# Autodesk Inventor assembly: Behavioural Device assembly
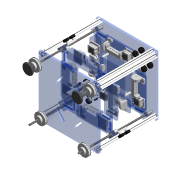
[picture p0: Inventor's stored thumbnail of the model, 180x180]
Saved by Autodesk Inventor 2020 (Build 240168000, 168)
## iProperties
Created: 2020-08-17
Part Number: Behavioural Device assembly
Document SubType Name: Assembly
Designer: ferrerx
Author: ferrerx
## Documents named in this file (22)
- C:\Users\ferrerx\Desktop\Prieto-Godino Lab\Drosophila Larvae Behavioural Device\Device design V3\Inventor Assembly\Behavioural Device assembly.iam
- C:\Users\ferrerx\Desktop\Inverted pendulum\aluminum profile.ipt
- C:\Users\ferrerx\Desktop\Prieto-Godino Lab\Drosophila Larvae Behavioural Device\Device design V3\Inventor Assembly\Z stage Base.ipt
- C:\Users\ferrerx\Desktop\Prieto-Godino Lab\Drosophila Larvae Behavioural Device\Device design V3\Inventor Assembly\Cart.ipt
- C:\Users\ferrerx\Desktop\Prieto-Godino Lab\Drosophila Larvae Behavioural Device\Device design V3\Inventor Assembly\Big pulley.ipt
- C:\Users\ferrerx\Desktop\Prieto-Godino Lab\Drosophila Larvae Behavioural Device\Device design V3\Inventor Assembly\guide wheel.ipt
- C:\Users\ferrerx\Desktop\Prieto-Godino Lab\Drosophila Larvae Behavioural Device\Device design V3\Inventor Assembly\Shaft connector.ipt
- C:\Users\ferrerx\Desktop\Prieto-Godino Lab\Drosophila Larvae Behavioural Device\Device design V3\Inventor Assembly\cart_spacer.ipt
- C:\Users\ferrerx\Desktop\Prieto-Godino Lab\Drosophila Larvae Behavioural Device\Device design V3\Inventor Assembly\Lead screw.ipt
- C:\Users\ferrerx\Desktop\Prieto-Godino Lab\Drosophila Larvae Behavioural Device\Device design V3\Inventor Assembly\lead screw nut.ipt
- C:\Users\ferrerx\Desktop\Prieto-Godino Lab\Drosophila Larvae Behavioural Device\Device design V3\Inventor Assembly\Light sources platform.ipt
- C:\Users\ferrerx\Desktop\Prieto-Godino Lab\Drosophila Larvae Behavioural Device\Device design V3\Inventor Assembly\Lead screw manual adjuster.ipt
- C:\Users\ferrerx\Desktop\Prieto-Godino Lab\Drosophila Larvae Behavioural Device\Device design V3\Inventor Assembly\Z stage Roof 2.ipt
- C:\Users\ferrerx\Desktop\Prieto-Godino Lab\Drosophila Larvae Behavioural Device\Device design V3\Inventor Assembly\Arena.ipt
- C:\Users\ferrerx\Desktop\Prieto-Godino Lab\Drosophila Larvae Behavioural Device\Device design V3\Inventor Assembly\Arena spacer.ipt
- C:\Users\ferrerx\Desktop\Prieto-Godino Lab\Drosophila Larvae Behavioural Device\Device design V3\Inventor Assembly\IR linear array assembly.iam
- C:\Users\ferrerx\Desktop\Prieto-Godino Lab\Drosophila Larvae Behavioural Device\Device design V3\Inventor Assembly\RGB matrices assembly.iam
- C:\Users\ferrerx\Desktop\Prieto-Godino Lab\Drosophila Larvae Behavioural Device\Device design V3\Inventor Assembly\Linear actuator assem 1.iam
- C:\Users\ferrerx\Desktop\Prieto-Godino Lab\Drosophila Larvae Behavioural Device\Device design V3\Inventor Assembly\pi_camera.ipt
- C:\Users\ferrerx\Desktop\Prieto-Godino Lab\Drosophila Larvae Behavioural Device\Device design V3\Inventor Assembly\Belt.ipt
- C:\Users\ferrerx\Desktop\Prieto-Godino Lab\Drosophila Larvae Behavioural Device\Device design V3\Inventor Assembly\LED Matrix Dotstar.ipt
- C:\Users\ferrerx\Desktop\Prieto-Godino Lab\Drosophila Larvae Behavioural Device\Device design V3\Inventor Assembly\LED Matrix 8X8.ipt
## Components (89 placed, 21 different names)
1. aluminum profile:1 — Mate:7, Mate:8, Mate:9, Mate:102, Mate:103, Mate:104, Angle:2, Angle:3
2. aluminum profile:2 — Mate:1, Mate:2, Mate:3, Angle:5
3. Z stage Base:2 — Mate:1, Mate:2, Mate:3, Mate:4, Mate:5, Mate:6, Mate:7, Mate:8, Mate:9, Mate:10, Mate:11, Mate:12, Mate:75, Mate:76, Mate:77, Mate:78, Mate:145, Mate:146, Mate:147, Mate:148, Mate:172, Mate:173, Mate:174, Mate:175, Mate:243, Mate:244
4. aluminum profile:3 — Mate:10, Mate:11, Mate:12, Angle:4
5. aluminum profile:4 — Mate:4, Mate:5, Mate:6, Angle:1, Angle:6
6. Cart:1 — Mate:45, Mate:46, Mate:47, Mate:48, Mate:49, Mate:50, Mate:52, Mate:53, Mate:69, Mate:70, Mate:87, Angle:4, Mate:196
7. Cart:2 — Mate:56, Mate:57, Mate:58, Mate:59, Mate:61, Mate:62, Mate:63, Mate:64, Mate:71, Mate:72, Mate:89, Mate:195, Angle:5
8. Big pulley:1 — Mate:95, Mate:106
9. Big pulley:2 — Mate:94, Mate:105, Mate:251, Mate:252
10. guide wheel:1 — Mate:29, Mate:55
11. guide wheel:2 — Mate:37, Mate:38
12. guide wheel:3 — Mate:44, Mate:60
13. guide wheel:4 — Mate:31, Mate:80
14. guide wheel:5 — Mate:32, Mate:51
15. guide wheel:6 — Mate:40, Mate:42
16. guide wheel:7 — Mate:30, Mate:54
17. guide wheel:8 — Mate:41, Mate:43
18. Shaft connector:1 — Mate:75, Mate:76, Mate:79, Mate:81
19. Shaft connector:2 — Mate:77, Mate:78, Mate:82, Mate:83
20. cart_spacer:1 — Mate:41, Mate:43, Mate:57, Mate:61
21. cart_spacer:2 — Mate:40, Mate:42, Mate:56, Mate:62
22. cart_spacer:3 — Mate:37, Mate:38, Mate:58, Mate:63
23. cart_spacer:4 — Mate:44, Mate:59, Mate:60, Mate:64
24. cart_spacer:5 — Mate:30, Mate:46, Mate:53, Mate:54
25. cart_spacer:6 — Mate:29, Mate:45, Mate:49, Mate:55
26. cart_spacer:7 — Mate:32, Mate:48, Mate:51, Mate:52
27. cart_spacer:8 — Mate:31, Mate:47, Mate:50, Mate:80
28. lead screw nut:3 — Mate:69, Mate:70, Mate:73, Mate:87
29. lead screw nut:4 — Mate:71, Mate:72, Mate:74, Mate:89
30. Lead screw:3 — Mate:73, Mate:79, Mate:81, Mate:94, Mate:99, Mate:100
31. Lead screw:4 — Mate:74, Mate:82, Mate:83, Mate:95
32. Light sources platform:1 — Mate:197, Mate:198, Mate:199, Mate:200, Mate:201, Mate:202, Mate:203, Mate:204, Mate:205, Mate:206, Mate:207, Mate:208, Mate:209, Angle:6, Mate:210, Mate:211
33. Lead screw manual adjuster:2 — Mate:99, Mate:100
34. Z stage Roof 2:1 — Mate:102, Mate:103, Mate:104, Mate:105, Mate:106, Mate:245, Mate:246, Mate:272
35. Lead screw:5 — Mate:149, Mate:151, Mate:154, Mate:156, Mate:157, Mate:161, Mate:180, Mate:209
36. Lead screw:6 — Mate:150, Mate:152, Mate:153, Mate:179
37. guide wheel:9 — Mate:116, Mate:117
38. guide wheel:10 — Mate:118, Mate:120
39. guide wheel:11 — Mate:119, Mate:121
40. guide wheel:12 — Mate:115, Mate:122
41. guide wheel:13 — Mate:134, Mate:138
42. guide wheel:14 — Mate:132, Mate:136
43. guide wheel:15 — Mate:133, Mate:137
44. guide wheel:16 — Mate:131, Mate:135
45. cart_spacer:9 — Mate:123, Mate:129, Mate:131, Mate:135
46. cart_spacer:10 — Mate:124, Mate:128, Mate:132, Mate:136
47. cart_spacer:11 — Mate:125, Mate:127, Mate:133, Mate:137
48. cart_spacer:12 — Mate:126, Mate:130, Mate:134, Mate:138
49. cart_spacer:13 — Mate:107, Mate:111, Mate:116, Mate:117
50. cart_spacer:14 — Mate:108, Mate:114, Mate:118, Mate:120
51. cart_spacer:15 — Mate:109, Mate:113, Mate:119, Mate:121
52. cart_spacer:16 — Mate:110, Mate:112, Mate:115, Mate:122
53. Cart:3 — Mate:123, Mate:124, Mate:125, Mate:126, Mate:127, Mate:128, Mate:129, Mate:130, Mate:141, Mate:142, Mate:143, Mate:179, Angle:2, Mate:211
54. Cart:4 — Mate:107, Mate:108, Mate:109, Mate:110, Mate:111, Mate:112, Mate:113, Mate:114, Mate:139, Mate:140, Mate:144, Angle:1, Mate:210
55. Light sources platform:2 — Mate:180, Angle:3, Mate:183, Mate:184, Mate:185, Mate:186, Mate:187, Mate:188, Mate:189, Mate:190, Mate:191, Mate:192, Mate:193, Mate:194, Mate:195, Mate:196
56. lead screw nut:5 — Mate:139, Mate:140, Mate:144, Mate:161
57. lead screw nut:6 — Mate:141, Mate:142, Mate:143
58. Lead screw manual adjuster:3 — Mate:156, Mate:157, Mate:160
59. Big pulley:3 — Mate:154, Mate:160, Mate:253, Mate:254
60. Big pulley:4 — Mate:153
61. Shaft connector:3 — Mate:145, Mate:148, Mate:150, Mate:152
62. Shaft connector:4 — Mate:146, Mate:147, Mate:149, Mate:151
63. Arena:1 — Mate:176, Mate:177, Mate:178, Mate:241, Mate:242, Mate:255, Mate:256, Mate:257, Mate:258, Mate:259, Mate:260, Mate:261, Mate:262, Mate:271
64. Arena spacer:1 — Mate:172, Mate:177, Mate:178
65. Arena spacer:2 — Mate:173, Mate:176, Mate:243
66. Arena spacer:3 — Mate:175, Mate:242
67. Arena spacer:4 — Mate:174, Mate:241, Mate:244
68. IR linear array assembly:1 [sub-assembly] — Mate:186, Mate:189, Mate:190
69. IR linear array assembly:2 [sub-assembly] — Mate:188, Mate:193, Mate:194
70. IR linear array assembly:3 [sub-assembly] — Mate:187, Mate:191, Mate:192
71. IR linear array assembly:4 [sub-assembly] — Mate:183, Mate:184, Mate:185
72. RGB matrices assembly:1 [sub-assembly] — Mate:203, Mate:204, Mate:205, Mate:266, Angle:7
73. RGB matrices assembly:2 [sub-assembly] — Mate:200, Mate:201, Mate:202, Mate:267, Angle:8
74. RGB matrices assembly:3 [sub-assembly] — Mate:197, Mate:198, Mate:199, Mate:268, Angle:9
75. RGB matrices assembly:4 [sub-assembly] — Mate:206, Mate:207, Mate:208, Mate:269, Angle:10, Mate:270
76. Linear actuator assem 1:1 [sub-assembly] — Mate:245, Mate:246, Mate:248, Mate:249, Mate:250, Mate:272
77. pi_camera:1 — Mate:248, Mate:249, Mate:250
78. Belt:1 — Mate:251, Mate:252
79. Belt:2 — Mate:253, Mate:254
80. Arena spacer:5 — Mate:258, Mate:261, Mate:264, Mate:265
81. Arena spacer:6 — Mate:256, Mate:260, Mate:263
82. Arena spacer:7 — Mate:255, Mate:259
83. Arena spacer:8 — Mate:257, Mate:262
84. Arena:2 — Mate:263, Mate:264, Mate:265
85. LED Matrix Dotstar:1 — Mate:267, Angle:8
86. LED Matrix Dotstar:2 — Mate:268, Angle:9
87. LED Matrix Dotstar:3 — Mate:266, Angle:7
88. LED Matrix Dotstar:4 — Mate:269, Angle:10, Mate:270
89. LED Matrix 8X8:1 — Mate:271
## Relationships (200: Mate 190, Angle 10)
- Mate:1: aluminum profile:2 ↔ Z stage Base:2
- Mate:2: aluminum profile:2 ↔ Z stage Base:2
- Mate:3: aluminum profile:2 ↔ Z stage Base:2
- Mate:4: Z stage Base:2 ↔ aluminum profile:4
- Mate:5: Z stage Base:2 ↔ aluminum profile:4
- Mate:6: Z stage Base:2 ↔ aluminum profile:4
- Mate:7: aluminum profile:1 ↔ Z stage Base:2
- Mate:8: aluminum profile:1 ↔ Z stage Base:2
- Mate:9: aluminum profile:1 ↔ Z stage Base:2
- Mate:10: Z stage Base:2 ↔ aluminum profile:3
- Mate:11: Z stage Base:2 ↔ aluminum profile:3
- Mate:12: Z stage Base:2 ↔ aluminum profile:3
- Mate:29: guide wheel:1 ↔ cart_spacer:6
- Mate:30: guide wheel:7 ↔ cart_spacer:5
- Mate:31: guide wheel:4 ↔ cart_spacer:8
- Mate:32: guide wheel:5 ↔ cart_spacer:7
- Mate:37: guide wheel:2 ↔ cart_spacer:3
- Mate:38: guide wheel:2 ↔ cart_spacer:3
- Mate:40: guide wheel:6 ↔ cart_spacer:2
- Mate:41: guide wheel:8 ↔ cart_spacer:1
- Mate:42: guide wheel:6 ↔ cart_spacer:2
- Mate:43: guide wheel:8 ↔ cart_spacer:1
- Mate:44: guide wheel:3 ↔ cart_spacer:4
- Mate:45: Cart:1 ↔ cart_spacer:6
- Mate:46: Cart:1 ↔ cart_spacer:5
- Mate:47: Cart:1 ↔ cart_spacer:8
- Mate:48: Cart:1 ↔ cart_spacer:7
- Mate:49: Cart:1 ↔ cart_spacer:6
- Mate:50: Cart:1 ↔ cart_spacer:8
- Mate:51: guide wheel:5 ↔ cart_spacer:7
- Mate:52: Cart:1 ↔ cart_spacer:7
- Mate:53: Cart:1 ↔ cart_spacer:5
- Mate:54: guide wheel:7 ↔ cart_spacer:5
- Mate:55: guide wheel:1 ↔ cart_spacer:6
- Mate:56: Cart:2 ↔ cart_spacer:2
- Mate:57: Cart:2 ↔ cart_spacer:1
- Mate:58: Cart:2 ↔ cart_spacer:3
- Mate:59: Cart:2 ↔ cart_spacer:4
- Mate:60: guide wheel:3 ↔ cart_spacer:4
- Mate:61: Cart:2 ↔ cart_spacer:1
- Mate:62: Cart:2 ↔ cart_spacer:2
- Mate:63: Cart:2 ↔ cart_spacer:3
- Mate:64: Cart:2 ↔ cart_spacer:4
- Mate:69: Cart:1 ↔ lead screw nut:3
- Mate:70: Cart:1 ↔ lead screw nut:3
- Mate:71: Cart:2 ↔ lead screw nut:4
- Mate:72: Cart:2 ↔ lead screw nut:4
- Mate:73: lead screw nut:3 ↔ Lead screw:3
- Mate:74: lead screw nut:4 ↔ Lead screw:4
- Mate:75: Z stage Base:2 ↔ Shaft connector:1
- Mate:76: Z stage Base:2 ↔ Shaft connector:1
- Mate:77: Z stage Base:2 ↔ Shaft connector:2
- Mate:78: Z stage Base:2 ↔ Shaft connector:2
- Mate:79: Shaft connector:1 ↔ Lead screw:3
- Mate:80: guide wheel:4 ↔ cart_spacer:8
- Mate:81: Shaft connector:1 ↔ Lead screw:3
- Mate:82: Shaft connector:2 ↔ Lead screw:4
- Mate:83: Shaft connector:2 ↔ Lead screw:4
- Mate:87: Cart:1 ↔ lead screw nut:3
- Mate:89: Cart:2 ↔ lead screw nut:4
- Mate:94: Big pulley:2 ↔ Lead screw:3
- Mate:95: Big pulley:1 ↔ Lead screw:4
- Mate:99: Lead screw:3 ↔ Lead screw manual adjuster:2
- Mate:100: Lead screw:3 ↔ Lead screw manual adjuster:2
- Mate:102: aluminum profile:1 ↔ Z stage Roof 2:1
- Mate:103: aluminum profile:1 ↔ Z stage Roof 2:1
- Mate:104: aluminum profile:1 ↔ Z stage Roof 2:1
- Mate:105: Big pulley:2 ↔ Z stage Roof 2:1
- Mate:106: Big pulley:1 ↔ Z stage Roof 2:1
- Mate:107: cart_spacer:13 ↔ Cart:4
- Mate:108: cart_spacer:14 ↔ Cart:4
- Mate:109: cart_spacer:15 ↔ Cart:4
- Mate:110: cart_spacer:16 ↔ Cart:4
- Mate:111: cart_spacer:13 ↔ Cart:4
- Mate:112: cart_spacer:16 ↔ Cart:4
- Mate:113: cart_spacer:15 ↔ Cart:4
- Mate:114: cart_spacer:14 ↔ Cart:4
- Mate:115: guide wheel:12 ↔ cart_spacer:16
- Mate:116: guide wheel:9 ↔ cart_spacer:13
- Mate:117: guide wheel:9 ↔ cart_spacer:13
- Mate:118: guide wheel:10 ↔ cart_spacer:14
- Mate:119: guide wheel:11 ↔ cart_spacer:15
- Mate:120: guide wheel:10 ↔ cart_spacer:14
- Mate:121: guide wheel:11 ↔ cart_spacer:15
- Mate:122: guide wheel:12 ↔ cart_spacer:16
- Mate:123: cart_spacer:9 ↔ Cart:3
- Mate:124: cart_spacer:10 ↔ Cart:3
- Mate:125: cart_spacer:11 ↔ Cart:3
- Mate:126: cart_spacer:12 ↔ Cart:3
- Mate:127: cart_spacer:11 ↔ Cart:3
- Mate:128: cart_spacer:10 ↔ Cart:3
- Mate:129: cart_spacer:9 ↔ Cart:3
- Mate:130: cart_spacer:12 ↔ Cart:3
- Mate:131: guide wheel:16 ↔ cart_spacer:9
- Mate:132: guide wheel:14 ↔ cart_spacer:10
- Mate:133: guide wheel:15 ↔ cart_spacer:11
- Mate:134: guide wheel:13 ↔ cart_spacer:12
- Mate:135: guide wheel:16 ↔ cart_spacer:9
- Mate:136: guide wheel:14 ↔ cart_spacer:10
- Mate:137: guide wheel:15 ↔ cart_spacer:11
- Mate:138: guide wheel:13 ↔ cart_spacer:12
- Mate:139: Cart:4 ↔ lead screw nut:5
- Mate:140: Cart:4 ↔ lead screw nut:5
- Mate:141: Cart:3 ↔ lead screw nut:6
- Mate:142: Cart:3 ↔ lead screw nut:6
- Mate:143: Cart:3 ↔ lead screw nut:6
- Mate:144: Cart:4 ↔ lead screw nut:5
- Mate:145: Z stage Base:2 ↔ Shaft connector:3
- Mate:146: Z stage Base:2 ↔ Shaft connector:4
- Mate:147: Z stage Base:2 ↔ Shaft connector:4
- Mate:148: Z stage Base:2 ↔ Shaft connector:3
- Mate:149: Lead screw:5 ↔ Shaft connector:4
- Mate:150: Lead screw:6 ↔ Shaft connector:3
- Mate:151: Lead screw:5 ↔ Shaft connector:4
- Mate:152: Lead screw:6 ↔ Shaft connector:3
- Mate:153: Lead screw:6 ↔ Big pulley:4
- Mate:154: Lead screw:5 ↔ Big pulley:3
- Mate:156: Lead screw:5 ↔ Lead screw manual adjuster:3
- Mate:157: Lead screw:5 ↔ Lead screw manual adjuster:3
- Mate:160: Lead screw manual adjuster:3 ↔ Big pulley:3
- Mate:161: Lead screw:5 ↔ lead screw nut:5
- Angle:1 (0 deg): aluminum profile:4 ↔ Cart:4
- Mate:172: Z stage Base:2 ↔ Arena spacer:1
- Mate:173: Z stage Base:2 ↔ Arena spacer:2
- Mate:174: Z stage Base:2 ↔ Arena spacer:4
- Mate:175: Z stage Base:2 ↔ Arena spacer:3
- Mate:176: Arena:1 ↔ Arena spacer:2
- Mate:177: Arena:1 ↔ Arena spacer:1
- Mate:178: Arena:1 ↔ Arena spacer:1
- Mate:179: Lead screw:6 ↔ Cart:3
- Angle:2 (0 deg): aluminum profile:1 ↔ Cart:3
- Mate:180: Lead screw:5 ↔ Light sources platform:2
- Angle:3 (0 deg): aluminum profile:1 ↔ Light sources platform:2
- Mate:183: Light sources platform:2 ↔ IR linear array assembly:4
- Mate:184: Light sources platform:2 ↔ IR linear array assembly:4
- Mate:185: Light sources platform:2 ↔ IR linear array assembly:4
- Mate:186: Light sources platform:2 ↔ IR linear array assembly:1
- Mate:187: Light sources platform:2 ↔ IR linear array assembly:3
- Mate:188: Light sources platform:2 ↔ IR linear array assembly:2
- Mate:189: Light sources platform:2 ↔ IR linear array assembly:1
- Mate:190: Light sources platform:2 ↔ IR linear array assembly:1
- Mate:191: Light sources platform:2 ↔ IR linear array assembly:3
- Mate:192: Light sources platform:2 ↔ IR linear array assembly:3
- Mate:193: Light sources platform:2 ↔ IR linear array assembly:2
- Mate:194: Light sources platform:2 ↔ IR linear array assembly:2
- Angle:4 (0 deg): aluminum profile:3 ↔ Cart:1
- Mate:195: Cart:2 ↔ Light sources platform:2
- Angle:5 (0 deg): aluminum profile:2 ↔ Cart:2
- Mate:196: Cart:1 ↔ Light sources platform:2
- Mate:197: Light sources platform:1 ↔ RGB matrices assembly:3
- Mate:198: Light sources platform:1 ↔ RGB matrices assembly:3
- Mate:199: Light sources platform:1 ↔ RGB matrices assembly:3
- Mate:200: Light sources platform:1 ↔ RGB matrices assembly:2
- Mate:201: Light sources platform:1 ↔ RGB matrices assembly:2
- Mate:202: Light sources platform:1 ↔ RGB matrices assembly:2
- Mate:203: Light sources platform:1 ↔ RGB matrices assembly:1
- Mate:204: Light sources platform:1 ↔ RGB matrices assembly:1
- Mate:205: Light sources platform:1 ↔ RGB matrices assembly:1
- Mate:206: Light sources platform:1 ↔ RGB matrices assembly:4
- Mate:207: Light sources platform:1 ↔ RGB matrices assembly:4
- Mate:208: Light sources platform:1 ↔ RGB matrices assembly:4
- Mate:209: Light sources platform:1 ↔ Lead screw:5
- Angle:6 (0 deg): aluminum profile:4 ↔ Light sources platform:1
- Mate:210: Light sources platform:1 ↔ Cart:4
- Mate:211: Light sources platform:1 ↔ Cart:3
- Mate:241: Arena:1 ↔ Arena spacer:4
- Mate:242: Arena:1 ↔ Arena spacer:3
- Mate:243: Z stage Base:2 ↔ Arena spacer:2
- Mate:244: Z stage Base:2 ↔ Arena spacer:4
- Mate:245: Z stage Roof 2:1 ↔ Linear actuator assem 1:1
- Mate:246: Z stage Roof 2:1 ↔ Linear actuator assem 1:1
- Mate:248: Linear actuator assem 1:1 ↔ pi_camera:1
- Mate:249: Linear actuator assem 1:1 ↔ pi_camera:1
- Mate:250: Linear actuator assem 1:1 ↔ pi_camera:1
- Mate:251: Big pulley:2 ↔ Belt:1
- Mate:252 (1 mm): Big pulley:2 ↔ Belt:1
- Mate:253: Big pulley:3 ↔ Belt:2
- Mate:254 (1 mm): Big pulley:3 ↔ Belt:2
- Mate:255: Arena:1 ↔ Arena spacer:7
- Mate:256: Arena:1 ↔ Arena spacer:6
- Mate:257: Arena:1 ↔ Arena spacer:8
- Mate:258: Arena:1 ↔ Arena spacer:5
- Mate:259: Arena:1 ↔ Arena spacer:7
- Mate:260: Arena:1 ↔ Arena spacer:6
- Mate:261: Arena:1 ↔ Arena spacer:5
- Mate:262: Arena:1 ↔ Arena spacer:8
- Mate:263: Arena spacer:6 ↔ Arena:2
- Mate:264: Arena spacer:5 ↔ Arena:2
- Mate:265: Arena spacer:5 ↔ Arena:2
- Mate:266: RGB matrices assembly:1 ↔ LED Matrix Dotstar:3
- Angle:7 (0 deg): RGB matrices assembly:1 ↔ LED Matrix Dotstar:3
- Mate:267: RGB matrices assembly:2 ↔ LED Matrix Dotstar:1
- Angle:8 (0 deg): RGB matrices assembly:2 ↔ LED Matrix Dotstar:1
- Mate:268: RGB matrices assembly:3 ↔ LED Matrix Dotstar:2
- Angle:9 (0 deg): RGB matrices assembly:3 ↔ LED Matrix Dotstar:2
- Mate:269: RGB matrices assembly:4 ↔ LED Matrix Dotstar:4
- Angle:10 (0 deg): RGB matrices assembly:4 ↔ LED Matrix Dotstar:4
- Mate:270: RGB matrices assembly:4 ↔ LED Matrix Dotstar:4
- Mate:271: Arena:1 ↔ LED Matrix 8X8:1
- Mate:272: Z stage Roof 2:1 ↔ Linear actuator assem 1:1
